# Autodesk Inventor assembly: Ensamble Pinza
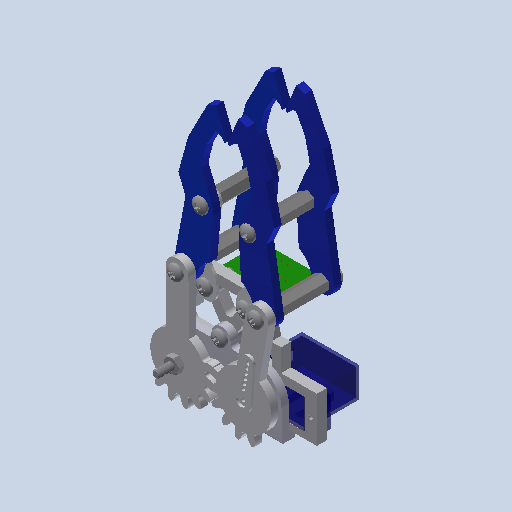
[picture p0: Inventor's stored thumbnail of the model, 512x512]
Saved by Autodesk Inventor 2022 (Build 260153000, 153)
## iProperties
Created: 2016-01-14
Part Number: Ensamble Pinza
Document SubType Name: Assembly
Designer: Nanjar
Author: Nanjar
## Documents named in this file (16)
- C:\Users\Administrador\Desktop\Octavo Semestre\Robótica Industrial\Robot\Pinza\Ensamble Pinza.iam
- C:\Users\Administrador\Desktop\Octavo Semestre\Robótica Industrial\Robot\Pinza\Partes\servo 9.ipt
- C:\Users\Administrador\Desktop\Octavo Semestre\Robótica Industrial\Robot\Pinza\Partes\gear2.ipt
- C:\Users\Administrador\Desktop\Octavo Semestre\Robótica Industrial\Robot\Pinza\Partes\gear2b.ipt
- C:\Users\Administrador\Desktop\Octavo Semestre\Robótica Industrial\Robot\Pinza\Partes\sheet_a.ipt
- C:\Users\Administrador\Desktop\Octavo Semestre\Robótica Industrial\Robot\Pinza\Partes\Part4.ipt
- C:\Users\Administrador\Desktop\Octavo Semestre\Robótica Industrial\Robot\Pinza\Partes\A1.ipt
- C:\Users\Administrador\Desktop\Octavo Semestre\Robótica Industrial\Robot\Pinza\Partes\arm1.ipt
- C:\Users\Administrador\Desktop\Octavo Semestre\Robótica Industrial\Robot\Pinza\Partes\arm1b.ipt
- C:\Users\Administrador\Desktop\Octavo Semestre\Robótica Industrial\Robot\Pinza\Partes\10Screw92005A120.ipt
- C:\Users\Administrador\Desktop\Octavo Semestre\Robótica Industrial\Robot\Pinza\Partes\Nut90591A121.ipt
- C:\Users\Administrador\Desktop\Octavo Semestre\Robótica Industrial\Robot\Pinza\Partes\20Screw92005A128.ipt
- C:\Users\Administrador\Desktop\Octavo Semestre\Robótica Industrial\Robot\Pinza\Partes\sheet4.ipt
- C:\Users\Administrador\Desktop\Octavo Semestre\Robótica Industrial\Robot\Pinza\Partes\grip1b - Can.ipt
- C:\Users\Administrador\Desktop\Octavo Semestre\Robótica Industrial\Robot\Pinza\Partes\spacer 19mm.ipt
- C:\Users\Administrador\Desktop\Octavo Semestre\Robótica Industrial\Robot\Pinza\Partes\PCB_Sen_Color.ipt
## Components (34 placed, 15 different names)
1. gear2:1 — Mate:1, Mate:2, Flush:1, Mate:5, Rotation:1, Mate:48, Mate:49, Mate:105, Mate:126
2. gear2b:1 — Mate:3, Mate:4, Flush:1, Mate:8, Mate:13, Rotation:1, Mate:113, Mate:115
3. servo 9:1 — Mate:5, Mate:6, Mate:7, Mate:9, Mate:10, Mate:11, Mate:13
4. sheet_a:1 — Mate:6, Mate:7, Mate:8, Mate:9, Mate:14, Mate:17, Mate:30, Mate:31, Mate:57, Mate:58, Mate:72, Mate:78, Mate:93, Mate:94
5. Part4:1 — Mate:10, Mate:11, Mate:12
6. A1:1 — Mate:12, Mate:48, Mate:49, Mate:71
7. arm1:1 — Mate:14, Mate:17, Mate:24, Mate:28, Mate:106, Mate:109, Mate:137
8. arm1b:1 — Mate:92, Mate:93, Mate:95, Mate:98, Mate:100, Mate:122
9. 10Screw92005A120:1 — Mate:24, Mate:28, Mate:29
10. 10Screw92005A120:3 — Mate:113, Mate:114, Mate:116
11. 10Screw92005A120:4 — Mate:26, Mate:92, Mate:94, Mate:95
12. Nut90591A121:1 — Mate:29, Mate:30
13. Nut90591A121:2 — Mate:26, Mate:31
14. 10Screw92005A120:5 — Mate:106, Mate:107, Mate:125, Mate:127
15. 10Screw92005A120:6 — Mate:98, Mate:101, Mate:120, Mate:121
16. Nut90591A121:6 — Mate:129, Mate:141
17. 10Screw92005A120:7 — Mate:52, Mate:105, Mate:108, Mate:126, Mate:128
18. Nut90591A121:7 — Mate:52, Mate:140
19. 20Screw92005A128:1 — Mate:57, Mate:58, Mate:70, Mate:142
20. sheet4:1 — Mate:70, Mate:71, Mate:72, Mate:76, Mate:77
21. 10Screw92005A120:8 — Mate:76, Mate:77, Mate:79
22. Nut90591A121:8 — Mate:78, Mate:79
23. grip1b - Can:1 — Mate:100, Mate:101, Mate:114, Mate:115, Mate:117, Mate:120
24. grip1b - Can:2 — Mate:107, Mate:108, Mate:109, Mate:125, Mate:139
25. spacer 19mm:1 — Mate:116, Mate:117, Mate:118, Mate:133, Mate:134
26. grip1b - Can:3 — Mate:118, Mate:123, Mate:124, Mate:135, Mate:136
27. spacer 19mm:2 — Mate:121, Mate:122, Mate:123, Mate:124, Mate:132
28. spacer 19mm:3 — Mate:128, Mate:130, Mate:139
29. spacer 19mm:4 — Mate:127, Mate:129, Mate:131, Mate:137, Mate:138
30. grip1b - Can:4 — Mate:130, Mate:131, Mate:138, Mate:140, Mate:141
31. Nut90591A121:9 — Mate:133, Mate:134, Mate:135
32. Nut90591A121:10 — Mate:132, Mate:136
33. Nut90591A121:11 — Mate:142
34. PCB_Sen_Color:1
## Relationships (76: Mate 74, Flush 1, RelateRotation 1)
- Mate:1: gear2:1
- Mate:2: gear2:1
- Mate:3 (26.26 mm): gear2b:1
- Mate:4: gear2b:1
- Flush:1: gear2:1 ↔ gear2b:1
- Mate:5: gear2:1 ↔ servo 9:1
- Mate:6: servo 9:1 ↔ sheet_a:1
- Mate:7: servo 9:1 ↔ sheet_a:1
- Mate:8: gear2b:1 ↔ sheet_a:1
- Mate:9: servo 9:1 ↔ sheet_a:1
- Mate:10: servo 9:1 ↔ Part4:1
- Mate:11: servo 9:1 ↔ Part4:1
- Mate:12: Part4:1 ↔ A1:1
- Mate:13: gear2b:1 ↔ servo 9:1
- Mate:14: sheet_a:1 ↔ arm1:1
- Mate:17: sheet_a:1 ↔ arm1:1
- Rotation:1 [RelateRotation] (1 ul): gear2:1 ↔ gear2b:1
- Mate:24: arm1:1 ↔ 10Screw92005A120:1
- Mate:26: 10Screw92005A120:4 ↔ Nut90591A121:2
- Mate:28: arm1:1 ↔ 10Screw92005A120:1
- Mate:29: 10Screw92005A120:1 ↔ Nut90591A121:1
- Mate:30: sheet_a:1 ↔ Nut90591A121:1
- Mate:31: sheet_a:1 ↔ Nut90591A121:2
- Mate:48: gear2:1 ↔ A1:1
- Mate:49: gear2:1 ↔ A1:1
- Mate:52: 10Screw92005A120:7 ↔ Nut90591A121:7
- Mate:57: sheet_a:1 ↔ 20Screw92005A128:1
- Mate:58: sheet_a:1 ↔ 20Screw92005A128:1
- Mate:70: 20Screw92005A128:1 ↔ sheet4:1
- Mate:71: A1:1 ↔ sheet4:1
- Mate:72: sheet_a:1 ↔ sheet4:1
- Mate:76: sheet4:1 ↔ 10Screw92005A120:8
- Mate:77: sheet4:1 ↔ 10Screw92005A120:8
- Mate:78: sheet_a:1 ↔ Nut90591A121:8
- Mate:79: 10Screw92005A120:8 ↔ Nut90591A121:8
- Mate:92: arm1b:1 ↔ 10Screw92005A120:4
- Mate:93: sheet_a:1 ↔ arm1b:1
- Mate:94: sheet_a:1 ↔ 10Screw92005A120:4
- Mate:95: arm1b:1 ↔ 10Screw92005A120:4
- Mate:98: arm1b:1 ↔ 10Screw92005A120:6
- Mate:100: arm1b:1 ↔ grip1b - Can:1
- Mate:101: 10Screw92005A120:6 ↔ grip1b - Can:1
- Mate:105: gear2:1 ↔ 10Screw92005A120:7
- Mate:106: arm1:1 ↔ 10Screw92005A120:5
- Mate:107: 10Screw92005A120:5 ↔ grip1b - Can:2
- Mate:108: 10Screw92005A120:7 ↔ grip1b - Can:2
- Mate:109: arm1:1 ↔ grip1b - Can:2
- Mate:113: gear2b:1 ↔ 10Screw92005A120:3
- Mate:114: 10Screw92005A120:3 ↔ grip1b - Can:1
- Mate:115: gear2b:1 ↔ grip1b - Can:1
- Mate:116: 10Screw92005A120:3 ↔ spacer 19mm:1
- Mate:117 (0.5 mm): grip1b - Can:1 ↔ spacer 19mm:1
- Mate:118: spacer 19mm:1 ↔ grip1b - Can:3
- Mate:120 (0.2 mm): 10Screw92005A120:6 ↔ grip1b - Can:1
- Mate:121: 10Screw92005A120:6 ↔ spacer 19mm:2
- Mate:122: arm1b:1 ↔ spacer 19mm:2
- Mate:123: grip1b - Can:3 ↔ spacer 19mm:2
- Mate:124: grip1b - Can:3 ↔ spacer 19mm:2
- Mate:125: 10Screw92005A120:5 ↔ grip1b - Can:2
- Mate:126: gear2:1 ↔ 10Screw92005A120:7
- Mate:127: 10Screw92005A120:5 ↔ spacer 19mm:4
- Mate:128: 10Screw92005A120:7 ↔ spacer 19mm:3
- Mate:129: Nut90591A121:6 ↔ spacer 19mm:4
- Mate:130: spacer 19mm:3 ↔ grip1b - Can:4
- Mate:131: spacer 19mm:4 ↔ grip1b - Can:4
- Mate:132: spacer 19mm:2 ↔ Nut90591A121:10
- Mate:133: spacer 19mm:1 ↔ Nut90591A121:9
- Mate:134: spacer 19mm:1 ↔ Nut90591A121:9
- Mate:135: grip1b - Can:3 ↔ Nut90591A121:9
- Mate:136: grip1b - Can:3 ↔ Nut90591A121:10
- Mate:137: arm1:1 ↔ spacer 19mm:4
- Mate:138: spacer 19mm:4 ↔ grip1b - Can:4
- Mate:139 (0.5 mm): grip1b - Can:2 ↔ spacer 19mm:3
- Mate:140: Nut90591A121:7 ↔ grip1b - Can:4
- Mate:141: Nut90591A121:6 ↔ grip1b - Can:4
- Mate:142: 20Screw92005A128:1 ↔ Nut90591A121:11
